# Autodesk Inventor assembly: HS 60T Gear, Square_MIR1
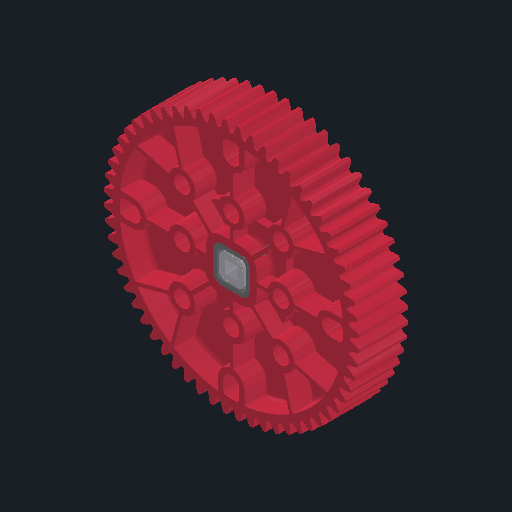
[picture p0: Inventor's stored thumbnail of the model, 512x512]
Saved by Autodesk Inventor 2023 (Build 270158000, 158)
## iProperties
Created: 2022-08-02
Part Number: HS 60T Gear, Square_MIR1
Document SubType Name: Assembly
Designer: Windows Macbook
Author: ylu12
## Documents named in this file (3)
- C:\Users\Windows Macbook\Desktop\VRC-SPIN-UP\Inventor\Motion\Gears\HS Gear\HS 60T Gear, Square_MIR1.iam
- C:\Users\Windows Macbook\Desktop\VRC-SPIN-UP\Inventor\Motion\HS Shaft Adapter Square_MIR1.ipt
- C:\Users\Windows Macbook\Desktop\VRC-SPIN-UP\Inventor\Motion\Gears\Reference Files\HS 60T Gear, No Insert_MIR1.ipt
## Components (2 placed, 2 different names)
1. HS Shaft Adapter Square_MIR1:1 — Flush:2, Mate:4, Mate:3
2. HS 60T Gear, No Insert_MIR1:1 — Mate:14, Mate:13, Flush:7
## Relationships (6: Mate 4, Flush 2)
- Flush:2 (-6.35 mm): HS Shaft Adapter Square_MIR1:1
- Mate:4: HS Shaft Adapter Square_MIR1:1
- Mate:3: HS Shaft Adapter Square_MIR1:1
- Mate:14: HS 60T Gear, No Insert_MIR1:1
- Mate:13: HS 60T Gear, No Insert_MIR1:1
- Flush:7: HS 60T Gear, No Insert_MIR1:1
